# Autodesk Inventor assembly: Landing_Gear
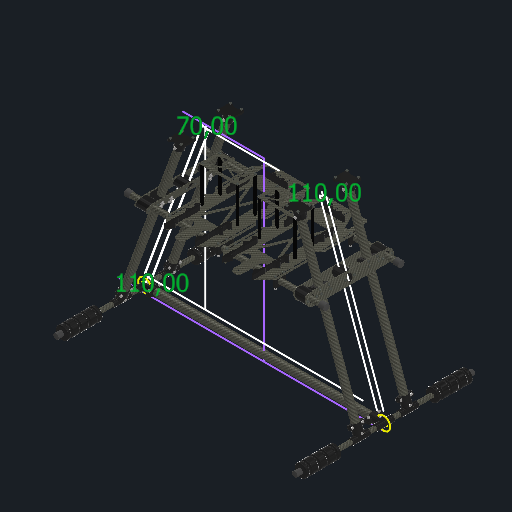
[picture p0: Inventor's stored thumbnail of the model, 512x512]
Saved by Autodesk Inventor 2025 (Build 290162010, 162A)
## iProperties
Created: 2023-12-07
Part Number: Landing_Gear
Document SubType Name: Assembly
Designer: dzw04
Mass: 1034.07 g
Surface Area: 7846.07 cm^2
Volume: 714.391 cm^3
Density: 1.44748 g/cm^3
Author: dzw04
## Documents named in this file (13)
- C:\Users\dhrzw\OneDrive - Saxion\Sarax_Pack_And_Go\Workspaces\Workspace\SARAX\01. CAD\01. 3D_Drawing\02. Sub_Assemblies\Landing_Gear\Landing_Gear.iam
- C:\Users\dhrzw\OneDrive - Saxion\Sarax_Pack_And_Go\Workspaces\Workspace\SARAX\01. CAD\01. 3D_Drawing\02. Sub_Assemblies\Landing_Gear\02. Sub_Assemblies\Leg_Frame_Connector_16mm.iam
- C:\Users\dhrzw\OneDrive - Saxion\Sarax_Pack_And_Go\Workspaces\Workspace\SARAX\01. CAD\01. 3D_Drawing\02. Sub_Assemblies\Landing_Gear\02. Sub_Assemblies\Leg_Feet_Connector_16-10mm.iam
- C:\Users\dhrzw\OneDrive - Saxion\Sarax_Pack_And_Go\Workspaces\Workspace\SARAX\01. CAD\01. 3D_Drawing\02. Sub_Assemblies\Landing_Gear\01. Parts\Landing_Gear_Feet.ipt
- C:\Users\dhrzw\OneDrive - Saxion\Sarax_Pack_And_Go\Workspaces\Workspace\SARAX\01. CAD\01. 3D_Drawing\02. Sub_Assemblies\Landing_Gear\01. Parts\10mm_Endcap.ipt
- C:\Users\dhrzw\OneDrive - Saxion\Sarax_Pack_And_Go\Workspaces\Workspace\SARAX\01. CAD\01. 3D_Drawing\02. Sub_Assemblies\Landing_Gear\01. Parts\Landing_Foam.ipt
- C:\Users\dhrzw\OneDrive - Saxion\Sarax_Pack_And_Go\Workspaces\Workspace\SARAX\01. CAD\01. 3D_Drawing\02. Sub_Assemblies\Landing_Gear\02. Sub_Assemblies\Leg_Loadpipe_Connector.iam
- C:\Users\dhrzw\OneDrive - Saxion\Sarax_Pack_And_Go\Workspaces\Workspace\SARAX\01. CAD\01. 3D_Drawing\02. Sub_Assemblies\Landing_Gear\01. Parts\12mm_Endcap.ipt
- C:\Users\dhrzw\OneDrive - Saxion\Sarax_Pack_And_Go\Workspaces\Workspace\SARAX\01. CAD\01. 3D_Drawing\02. Sub_Assemblies\Battery_Tray\Battery_Tray.iam
- C:\Users\dhrzw\OneDrive - Saxion\Sarax_Pack_And_Go\Workspaces\Workspace\SARAX\01. CAD\01. 3D_Drawing\02. Sub_Assemblies\Landing_Gear\01. Parts\Loadpipe.ipt
- C:\Users\dhrzw\OneDrive - Saxion\Sarax_Pack_And_Go\Workspaces\Workspace\SARAX\01. CAD\01. 3D_Drawing\02. Sub_Assemblies\Landing_Gear\01. Parts\Landing_Gear_Stability_Bar.ipt
- C:\Users\dhrzw\OneDrive - Saxion\Sarax_Pack_And_Go\Workspaces\Workspace\SARAX\01. CAD\01. 3D_Drawing\02. Sub_Assemblies\Landing_Gear\01. Parts\Landing_Gear_Rod.ipt
- C:\Users\dhrzw\OneDrive - Saxion\Sarax_Pack_And_Go\Workspaces\Workspace\SARAX\01. CAD\01. 3D_Drawing\Parameters.xlsx
## Components (35 placed, 11 different names)
1. Leg_Frame_Connector_16mm:1 [sub-assembly] — Flush:1, Mate:1, Flush:5, Flush:6, Mate:3, Mate:4, Mate:10, Mate:71
2. Leg_Frame_Connector_16mm:2 [sub-assembly] — Flush:1, Flush:2, Flush:3, Mate:1, Flush:5, Mate:5, Mate:11
3. Leg_Frame_Connector_16mm:3 [sub-assembly] — Flush:3, Mate:2, Flush:4, Mate:6, Mate:9
4. Leg_Frame_Connector_16mm:4 [sub-assembly] — Flush:2, Mate:2, Flush:4, Flush:6, Mate:3, Mate:7, Mate:8, Flush:12, Flush:14, Flush:15
5. Landing_Gear_Rod:1 — Mate:4, Mate:10, Mate:14, Mate:15, Mate:49
6. Landing_Gear_Rod:2 — Mate:5, Mate:11, Mate:12, Mate:13, Mate:50
7. Landing_Gear_Rod:3 — Mate:6, Mate:9, Mate:16, Mate:17, Mate:48
8. Landing_Gear_Rod:4 — Mate:7, Mate:8, Mate:18, Mate:19, Mate:47
9. Leg_Feet_Connector_16-10mm:1 [sub-assembly] — Mate:18, Mate:19, Mate:20, Flush:8
10. Leg_Feet_Connector_16-10mm:2 [sub-assembly] — Mate:16, Mate:17, Mate:21
11. Leg_Feet_Connector_16-10mm:3 [sub-assembly] — Mate:14, Mate:15, Mate:22
12. Leg_Feet_Connector_16-10mm:4 [sub-assembly] — Mate:12, Mate:13, Mate:23, Mate:74
13. Landing_Gear_Feet:1 — Mate:22, Mate:23, Flush:7, Mate:25, Mate:27, Mate:28, Mate:29, Mate:32, Mate:33, Mate:73
14. Landing_Gear_Feet:2 — Mate:20, Mate:21, Flush:7, Flush:8, Mate:24, Mate:26, Mate:30, Mate:31, Mate:34, Mate:35, Mate:75
15. 10mm_Endcap:1 — Mate:25, Mate:29, Mate:38
16. 10mm_Endcap:2 — Mate:26, Mate:30, Mate:36
17. 10mm_Endcap:3 — Mate:27, Mate:28, Mate:39
18. 10mm_Endcap:4 — Mate:24, Mate:31, Mate:37
19. Landing_Foam:1 — Mate:35, Mate:37
20. Landing_Foam:2 — Mate:34, Mate:36
21. Landing_Foam:3 — Mate:32, Mate:38
22. Landing_Foam:4 — Mate:33, Mate:39
23. Leg_Feet_Connector_16-10mm:5 [sub-assembly] — Mate:44, Mate:46, Mate:73, Mate:74
24. Leg_Feet_Connector_16-10mm:6 [sub-assembly] — Mate:72, Mate:75
25. Landing_Gear_Stability_Bar:1 — Mate:44, Mate:46, Mate:72
26. Leg_Loadpipe_Connector:1 [sub-assembly] — Mate:47, Mate:48, Flush:9, Mate:52, Mate:53, Flush:12
27. Leg_Loadpipe_Connector:2 [sub-assembly] — Mate:49, Mate:50, Flush:9, Mate:54, Mate:55
28. Loadpipe:5 — Mate:53, Mate:55, Flush:10, Flush:11, Mate:56, Mate:60, Mate:61, Mate:64, Mate:67
29. Loadpipe:6 — Mate:52, Mate:54, Flush:11, Mate:57, Mate:58, Mate:59, Mate:62, Mate:63, Mate:68, Flush:13
30. 12mm_Endcap:1 — Mate:62, Mate:63
31. 12mm_Endcap:2 — Mate:61, Mate:64
32. 12mm_Endcap:3 — Mate:57, Mate:58, Mate:59
33. 12mm_Endcap:4 — Mate:56, Mate:60
34. Battery_Tray:1 [sub-assembly] — Mate:65, Mate:66, Mate:69
35. Battery_Tray:2 [sub-assembly] — Mate:65, Mate:66, Mate:67, Mate:68, Mate:69, Flush:13
## Relationships (83: Mate 68, Flush 15)
- Flush:1: Leg_Frame_Connector_16mm:1 ↔ Leg_Frame_Connector_16mm:2
- Flush:2: Leg_Frame_Connector_16mm:2 ↔ Leg_Frame_Connector_16mm:4
- Flush:3: Leg_Frame_Connector_16mm:2 ↔ Leg_Frame_Connector_16mm:3
- Mate:1 (76 mm): Leg_Frame_Connector_16mm:1 ↔ Leg_Frame_Connector_16mm:2
- Mate:2 (76 mm): Leg_Frame_Connector_16mm:3 ↔ Leg_Frame_Connector_16mm:4
- Flush:4: Leg_Frame_Connector_16mm:3 ↔ Leg_Frame_Connector_16mm:4
- Flush:5: Leg_Frame_Connector_16mm:1 ↔ Leg_Frame_Connector_16mm:2
- Flush:6: Leg_Frame_Connector_16mm:1 ↔ Leg_Frame_Connector_16mm:4
- Mate:3 (232 mm): Leg_Frame_Connector_16mm:1 ↔ Leg_Frame_Connector_16mm:4
- Mate:4: Leg_Frame_Connector_16mm:1 ↔ Landing_Gear_Rod:1
- Mate:5: Leg_Frame_Connector_16mm:2 ↔ Landing_Gear_Rod:2
- Mate:6: Leg_Frame_Connector_16mm:3 ↔ Landing_Gear_Rod:3
- Mate:7: Leg_Frame_Connector_16mm:4 ↔ Landing_Gear_Rod:4
- Mate:8: Leg_Frame_Connector_16mm:4 ↔ Landing_Gear_Rod:4
- Mate:9: Leg_Frame_Connector_16mm:3 ↔ Landing_Gear_Rod:3
- Mate:10: Leg_Frame_Connector_16mm:1 ↔ Landing_Gear_Rod:1
- Mate:11: Leg_Frame_Connector_16mm:2 ↔ Landing_Gear_Rod:2
- Mate:12: Landing_Gear_Rod:2 ↔ Leg_Feet_Connector_16-10mm:4
- Mate:13: Landing_Gear_Rod:2 ↔ Leg_Feet_Connector_16-10mm:4
- Mate:14: Landing_Gear_Rod:1 ↔ Leg_Feet_Connector_16-10mm:3
- Mate:15: Landing_Gear_Rod:1 ↔ Leg_Feet_Connector_16-10mm:3
- Mate:16: Landing_Gear_Rod:3 ↔ Leg_Feet_Connector_16-10mm:2
- Mate:17: Landing_Gear_Rod:3 ↔ Leg_Feet_Connector_16-10mm:2
- Mate:18: Landing_Gear_Rod:4 ↔ Leg_Feet_Connector_16-10mm:1
- Mate:19: Landing_Gear_Rod:4 ↔ Leg_Feet_Connector_16-10mm:1
- Mate:20: Leg_Feet_Connector_16-10mm:1 ↔ Landing_Gear_Feet:2
- Mate:21: Leg_Feet_Connector_16-10mm:2 ↔ Landing_Gear_Feet:2
- Mate:22: Leg_Feet_Connector_16-10mm:3 ↔ Landing_Gear_Feet:1
- Mate:23: Leg_Feet_Connector_16-10mm:4 ↔ Landing_Gear_Feet:1
- Flush:7: Landing_Gear_Feet:1 ↔ Landing_Gear_Feet:2
- Flush:8 (-125 mm): Leg_Feet_Connector_16-10mm:1 ↔ Landing_Gear_Feet:2
- Mate:24: Landing_Gear_Feet:2 ↔ 10mm_Endcap:4
- Mate:25: Landing_Gear_Feet:1 ↔ 10mm_Endcap:1
- Mate:26: Landing_Gear_Feet:2 ↔ 10mm_Endcap:2
- Mate:27: Landing_Gear_Feet:1 ↔ 10mm_Endcap:3
- Mate:28: Landing_Gear_Feet:1 ↔ 10mm_Endcap:3
- Mate:29: Landing_Gear_Feet:1 ↔ 10mm_Endcap:1
- Mate:30: Landing_Gear_Feet:2 ↔ 10mm_Endcap:2
- Mate:31: Landing_Gear_Feet:2 ↔ 10mm_Endcap:4
- Mate:32: Landing_Gear_Feet:1 ↔ Landing_Foam:3
- Mate:33: Landing_Gear_Feet:1 ↔ Landing_Foam:4
- Mate:34: Landing_Gear_Feet:2 ↔ Landing_Foam:2
- Mate:35: Landing_Gear_Feet:2 ↔ Landing_Foam:1
- Mate:36: 10mm_Endcap:2 ↔ Landing_Foam:2
- Mate:37: 10mm_Endcap:4 ↔ Landing_Foam:1
- Mate:38: 10mm_Endcap:1 ↔ Landing_Foam:3
- Mate:39: 10mm_Endcap:3 ↔ Landing_Foam:4
- Mate:44: Leg_Feet_Connector_16-10mm:5 ↔ Landing_Gear_Stability_Bar:1
- Mate:46: Leg_Feet_Connector_16-10mm:5 ↔ Landing_Gear_Stability_Bar:1
- Mate:47: Landing_Gear_Rod:4 ↔ Leg_Loadpipe_Connector:1
- Mate:48: Landing_Gear_Rod:3 ↔ Leg_Loadpipe_Connector:1
- Mate:49: Landing_Gear_Rod:1 ↔ Leg_Loadpipe_Connector:2
- Mate:50: Landing_Gear_Rod:2 ↔ Leg_Loadpipe_Connector:2
- Flush:9: Leg_Loadpipe_Connector:1 ↔ Leg_Loadpipe_Connector:2
- Mate:52: Leg_Loadpipe_Connector:1 ↔ Loadpipe:6
- Mate:53: Leg_Loadpipe_Connector:1 ↔ Loadpipe:5
- Mate:54: Leg_Loadpipe_Connector:2 ↔ Loadpipe:6
- Mate:55: Leg_Loadpipe_Connector:2 ↔ Loadpipe:5
- Flush:10 (-225 mm): Loadpipe:5
- Flush:11: Loadpipe:5 ↔ Loadpipe:6
- Mate:56: Loadpipe:5 ↔ 12mm_Endcap:4
- Mate:57: Loadpipe:6 ↔ 12mm_Endcap:3
- Mate:58: Loadpipe:6 ↔ 12mm_Endcap:3
- Mate:59: Loadpipe:6 ↔ 12mm_Endcap:3
- Mate:60: Loadpipe:5 ↔ 12mm_Endcap:4
- Mate:61: Loadpipe:5 ↔ 12mm_Endcap:2
- Mate:62: Loadpipe:6 ↔ 12mm_Endcap:1
- Mate:63: Loadpipe:6 ↔ 12mm_Endcap:1
- Mate:64: Loadpipe:5 ↔ 12mm_Endcap:2
- Flush:12 (-126 mm): Leg_Frame_Connector_16mm:4 ↔ Leg_Loadpipe_Connector:1
- Mate:65: Battery_Tray:1 ↔ Battery_Tray:2
- Mate:66: Battery_Tray:1 ↔ Battery_Tray:2
- Mate:67: Loadpipe:5 ↔ Battery_Tray:2
- Mate:68: Loadpipe:6 ↔ Battery_Tray:2
- Mate:69 (10 mm): Battery_Tray:1 ↔ Battery_Tray:2
- Flush:13 (102.5 mm): Loadpipe:6 ↔ Battery_Tray:2
- Mate:71 (116 mm): Leg_Frame_Connector_16mm:1
- Flush:14: Leg_Frame_Connector_16mm:4
- Flush:15 (38 mm): Leg_Frame_Connector_16mm:4
- Mate:72: Leg_Feet_Connector_16-10mm:6 ↔ Landing_Gear_Stability_Bar:1
- Mate:73: Landing_Gear_Feet:1 ↔ Leg_Feet_Connector_16-10mm:5
- Mate:74 (15 mm): Leg_Feet_Connector_16-10mm:4 ↔ Leg_Feet_Connector_16-10mm:5
- Mate:75: Landing_Gear_Feet:2 ↔ Leg_Feet_Connector_16-10mm:6
## Named parameters: BatteryLength = 200 mm, BatteryWidth = 62 mm, BatteryHeight = 76 mm, NumberOfArms = 4, RotorToRotor = 900 mm, MountToMotorCenter = 0 mm, ArmPosition = 5 deg, ThicknessBodyCenterPlate = 2 mm, ThicknessBodyOuterPlate = 2 mm, ThicknessLegLoadpipePlate = 2 mm, ThicknessBatteryTray = 2 mm, ThicknessBatteryTopTray = 1 mm, LoadpipeLength = 450 mm, NumberOfBatterys = 2, LandingGearHeight = 400 mm, LandingGearStabilityBar = 525 mm, LandingGearRod = 390 mm, StartAngleArm = 45 deg, MotorMountCenter = 71.5 mm
